# Autodesk Inventor assembly: motor_assembly
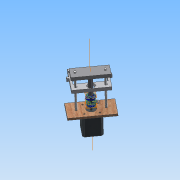
[picture p0: Inventor's stored thumbnail of the model, 180x180]
Saved by Autodesk Inventor 2015 (Build 190159000, 159)
## iProperties
Created: 2013-12-24
Part Number: motor_assembly
Document SubType Name: Assembly
Designer: aoki
Author: aoki
## Documents named in this file (9)
- C:\Users\shohei\Documents\Inventor\PlasmaCNCrev3\Workspaces\Workspace\main\motor_assembly_z.iam
- C:\Users\shohei\Documents\Inventor\PlasmaCNCrev3\Workspaces\Workspace\42BYGHM809.ipt
- C:\Users\shohei\Documents\Inventor\PlasmaCNCrev3\Workspaces\Workspace\main\TaperedNut.ipt
- C:\Users\shohei\Documents\Inventor\PlasmaCNCrev3\Workspaces\Workspace\main\TaperedScrewCoupling_8x5.ipt
- C:\Users\shohei\Documents\Inventor\PlasmaCNCrev3\Workspaces\Workspace\main\drive_schaft_8.ipt
- C:\Users\shohei\Documents\Inventor\PlasmaCNCrev3\Workspaces\Workspace\main\holder_schaft_9.ipt
- C:\Users\shohei\Documents\Inventor\PlasmaCNCrev3\Workspaces\Workspace\holder_plate2.ipt
- C:\Users\shohei\Documents\Inventor\PlasmaCNCrev3\Workspaces\Workspace\main\drieparts_assembly2.ipt
- C:\Users\shohei\Documents\Inventor\PlasmaCNCrev3\Workspaces\Workspace\theotherside.ipt
## Components (10 placed, 8 different names)
1. 42BYGHM809:1 — Insert:1, Mate:33, Mate:34, Mate:35
2. TaperedNut:1 — Rotational:1, Rigid:2
3. TaperedScrewCoupling_8x5:1 — Rotational:1, Insert:1
4. TaperedNut:2 — Rigid:2, Rigid:3
5. drive_schaft_8:1 — Rigid:3, Mate:1
6. holder_schaft_9:1 — Cylindrical:3, Flush:2, Cylindrical:5
7. holder_schaft_9:2 — Cylindrical:1, Flush:1, Cylindrical:4
8. holder_plate2:1 — Mate:33, Mate:34, Mate:35, Cylindrical:1, Cylindrical:3, Flush:1, Flush:2
9. drieparts_assembly2:1
10. theotherside:1 — Cylindrical:4, Cylindrical:5
## Relationships (14: Mate 4, CylindricalJoint 4, WeldJoint 2, Flush 2, RevoluteJoint 1, Insert 1)
- Rotational:1 [RevoluteJoint]: TaperedNut:1 ↔ TaperedScrewCoupling_8x5:1
- Rigid:2 [WeldJoint] (-15 mm): TaperedNut:1 ↔ TaperedNut:2
- Rigid:3 [WeldJoint] (-2.5 mm): TaperedNut:2 ↔ drive_schaft_8:1
- Mate:1: drive_schaft_8:1
- Insert:1 (-10 mm): 42BYGHM809:1 ↔ TaperedScrewCoupling_8x5:1
- Mate:33: 42BYGHM809:1 ↔ holder_plate2:1
- Mate:34: 42BYGHM809:1 ↔ holder_plate2:1
- Mate:35: 42BYGHM809:1 ↔ holder_plate2:1
- Cylindrical:1: holder_schaft_9:2 ↔ holder_plate2:1
- Cylindrical:3: holder_schaft_9:1 ↔ holder_plate2:1
- Flush:1: holder_schaft_9:2 ↔ holder_plate2:1
- Flush:2: holder_schaft_9:1 ↔ holder_plate2:1
- Cylindrical:4: holder_schaft_9:2 ↔ theotherside:1
- Cylindrical:5: holder_schaft_9:1 ↔ theotherside:1
